# Autodesk Inventor assembly: Assembly_Lens_Object_Mount
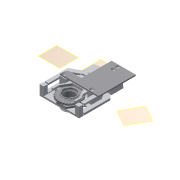
[picture p0: Inventor's stored thumbnail of the model, 180x180]
Saved by Autodesk Inventor 2016 (Build 200138000, 138)
## iProperties
Created: 2017-11-17
Part Number: Assembly_Lens_Object_Mount
Material: Generisch
Document SubType Name: Assembly
Designer: diederichbenedict
Author: diederichbenedict
## Documents named in this file (7)
- C:\Users\diederichbenedict\Dropbox\Dokumente\Promotion\PROJECTS\Beamerscope\Inventor\Beamerscope_r5\Assembly_Lens_Object_Mount.iam
- C:\Users\diederichbenedict\Dropbox\Dokumente\Promotion\PROJECTS\Beamerscope\Inventor\Beamerscope_r5\06_Case_Upper_v1.ipt
- C:\Users\diederichbenedict\Dropbox\Dokumente\Promotion\PROJECTS\Beamerscope\Inventor\Beamerscope_r5\27_Nut.ipt
- C:\Users\diederichbenedict\Dropbox\Dokumente\Promotion\PROJECTS\Beamerscope\Inventor\Beamerscope_r5\26_Lensholder_Aspheric_right.ipt
- C:\Users\diederichbenedict\Dropbox\Dokumente\Promotion\PROJECTS\Beamerscope\Inventor\Beamerscope_r5\28_Z_Stage.ipt
- C:\Users\diederichbenedict\Dropbox\Dokumente\Promotion\PROJECTS\Beamerscope\Inventor\Beamerscope_r5\11_Smartphone_Platform.ipt
- C:\Users\diederichbenedict\Dropbox\Dokumente\Promotion\PROJECTS\Beamerscope\Inventor\Beamerscope_r5\30_Nut_Gear.ipt
## Components (6 placed, 6 different names)
1. 06_Case_Upper_v1:1 — Winkel:1
2. 27_Nut:1 — Winkel:1
3. 26_Lensholder_Aspheric_right:1 — Einfügen:2
4. 28_Z_Stage:1
5. 11_Smartphone_Platform:1
6. 30_Nut_Gear:1 — Einfügen:2
## Relationships (3: Insert 2, Angle 1)
- [Insert] (-15 mm): 27_Nut:1 ↔ 26_Lensholder_Aspheric_right:1
- Winkel:1 [Angle] (0 deg): 06_Case_Upper_v1:1 ↔ 27_Nut:1
- Einfügen:2 [Insert] (5 mm): 26_Lensholder_Aspheric_right:1 ↔ 30_Nut_Gear:1
